# Autodesk Inventor assembly: Baugruppe_Christian_Test
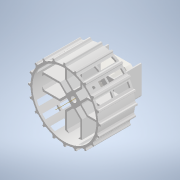
[picture p0: Inventor's stored thumbnail of the model, 180x180]
Saved by Autodesk Inventor 2021 (Build 250183000, 183)
## iProperties
Created: 2021-01-04
Part Number: Baugruppe_Christian_Test
Document SubType Name: Assembly
Designer: Ctroi
Author: Ctroi
## Documents named in this file (5)
- G:\Roverprojekt\Github Projekt\Rover\Baugruppe_Christian_Test.iam
- G:\Roverprojekt\Github Projekt\Rover\Motorhalterung_v2.ipt
- G:\Roverprojekt\Github Projekt\Rover\Steppermotor.ipt
- G:\Roverprojekt\Github Projekt\Rover\Reifen_v2.ipt
- G:\Roverprojekt\Github Projekt\Rover\Verbindung_Motor_Servo.ipt
## Components (4 placed, 4 different names)
1. Motorhalterung_v2:1 — Einfügen:1
2. Steppermotor:1 — Einfügen:1, Einfügen:2
3. Reifen_v2:1 — Einfügen:2
4. Verbindung_Motor_Servo:1
## Relationships (2: Insert 2)
- Einfügen:1 [Insert] (-20 mm): Motorhalterung_v2:1 ↔ Steppermotor:1
- Einfügen:2 [Insert] (-20 mm): Steppermotor:1 ↔ Reifen_v2:1
